# Autodesk Inventor assembly: LED Assembly
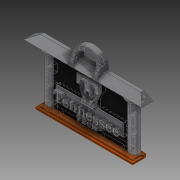
[picture p0: Inventor's stored thumbnail of the model, 180x180]
Saved by Autodesk Inventor 2018 (Build 220112000, 112)
## iProperties
Created: 2017-12-07
Part Number: LED Assembly
Document SubType Name: Assembly
Designer: Rus
Author: Rus
## Documents named in this file (10)
- E:\Libraries\Documents\3D Models\2017 TN Tech Ornament\Split\LED Assembly SPLIT.iam
- E:\Libraries\Documents\3D Models\2017 TN Tech Ornament\LED.ipt
- E:\Libraries\Documents\3D Models\2017 TN Tech Ornament\Split\3D Printed2 LED parent.ipt
- E:\Libraries\Documents\3D Models\2017 TN Tech Ornament\Split\3D Printed2 LED Pillar R white.ipt
- E:\Libraries\Documents\3D Models\2017 TN Tech Ornament\Split\3D Printed2 LED Top Grey.ipt
- E:\Libraries\Documents\3D Models\2017 TN Tech Ornament\Split\3D Printed2 LED Pillar L white 2.ipt
- E:\Libraries\Documents\3D Models\2017 TN Tech Ornament\Split\3D Printed2 LED Steps Brown.ipt
- E:\Libraries\Documents\3D Models\2017 TN Tech Ornament\Split\3D Printed2 LED Mid Black.ipt
- E:\Libraries\Documents\3D Models\2017 TN Tech Ornament\Split\3D Printed2 LED Text Bird.ipt
- E:\Libraries\Documents\3D Models\2017 TN Tech Ornament\Split\3D Printed2 LED Text text.ipt
## Components (18 placed, 9 different names)
1. LED:1 — Angle:2, Angle:18, Insert:1
2. 3D Printed2 LED parent:1 — Angle:2, Angle:3, Angle:4, Angle:5, Angle:6, Angle:7, Angle:8, Angle:9, Angle:10, Angle:11, Angle:12, Angle:13, Angle:14, Angle:15, Angle:16, Angle:17, Angle:18, Insert:1, Insert:2, Insert:3, Insert:4, Insert:5, Insert:6, Insert:7, Insert:8, Insert:9, Insert:10
3. LED:2 — Angle:4, Angle:16, Insert:4
4. LED:3 — Angle:5, Angle:15, Insert:2
5. LED:4 — Angle:3, Angle:17, Insert:6
6. LED:5 — Angle:9, Insert:9
7. LED:6 — Angle:7, Angle:13, Insert:3
8. LED:7 — Angle:8, Angle:11, Insert:7
9. LED:8 — Angle:6, Angle:14, Insert:8
10. LED:9 — Angle:10, Insert:5
11. LED:10 — Angle:12, Insert:10
12. 3D Printed2 LED Pillar R white:1 — Flush:2, Mate:1, Mate:3, Flush:3, Flush:4, Flush:6, Mate:8
13. 3D Printed2 LED Top Grey:1 — Flush:2, Mate:1, Mate:2, Angle:19, Mate:4, Mate:6, Angle:21, Mate:11, Angle:22, Mate:14
14. 3D Printed2 LED Pillar L white 2:1 — Flush:3, Flush:4, Mate:4, Flush:7, Flush:9
15. 3D Printed2 LED Steps Brown:1 — Flush:6, Mate:8, Flush:7
16. 3D Printed2 LED Mid Black:1 — Flush:8, Mate:9, Mate:10, Flush:9, Mate:12, Angle:23, Mate:14
17. 3D Printed2 LED Text Bird:1 — Flush:8, Mate:9, Mate:10
18. 3D Printed2 LED Text text:1
## Relationships (51: Angle 21, Mate 13, Insert 10, Flush 7)
- Angle:2 (0 deg): LED:1 ↔ 3D Printed2 LED parent:1
- Angle:3 (0 deg): 3D Printed2 LED parent:1 ↔ LED:4
- Angle:4 (0 deg): 3D Printed2 LED parent:1 ↔ LED:2
- Angle:5 (0 deg): 3D Printed2 LED parent:1 ↔ LED:3
- Angle:6 (0 deg): 3D Printed2 LED parent:1 ↔ LED:8
- Angle:7 (0 deg): 3D Printed2 LED parent:1 ↔ LED:6
- Angle:8 (0 deg): 3D Printed2 LED parent:1 ↔ LED:7
- Angle:9 (0 deg): 3D Printed2 LED parent:1 ↔ LED:5
- Angle:10 (0 deg): 3D Printed2 LED parent:1 ↔ LED:9
- Angle:11 (0 deg): 3D Printed2 LED parent:1 ↔ LED:7
- Angle:12 (0 deg): 3D Printed2 LED parent:1 ↔ LED:10
- Angle:13 (0 deg): 3D Printed2 LED parent:1 ↔ LED:6
- Angle:14 (0 deg): 3D Printed2 LED parent:1 ↔ LED:8
- Angle:15 (0 deg): 3D Printed2 LED parent:1 ↔ LED:3
- Angle:16 (0 deg): 3D Printed2 LED parent:1 ↔ LED:2
- Angle:17 (0 deg): 3D Printed2 LED parent:1 ↔ LED:4
- Angle:18 (0 deg): LED:1 ↔ 3D Printed2 LED parent:1
- Insert:1: LED:1 ↔ 3D Printed2 LED parent:1
- Insert:2: 3D Printed2 LED parent:1 ↔ LED:3
- Insert:3: 3D Printed2 LED parent:1 ↔ LED:6
- Insert:4: 3D Printed2 LED parent:1 ↔ LED:2
- Insert:5: 3D Printed2 LED parent:1 ↔ LED:9
- Insert:6: 3D Printed2 LED parent:1 ↔ LED:4
- Insert:7: 3D Printed2 LED parent:1 ↔ LED:7
- Insert:8: 3D Printed2 LED parent:1 ↔ LED:8
- Insert:9: 3D Printed2 LED parent:1 ↔ LED:5
- Insert:10: 3D Printed2 LED parent:1 ↔ LED:10
- Flush:2: 3D Printed2 LED Pillar R white:1 ↔ 3D Printed2 LED Top Grey:1
- Mate:1: 3D Printed2 LED Pillar R white:1 ↔ 3D Printed2 LED Top Grey:1
- Mate:2: 3D Printed2 LED Top Grey:1
- Angle:19 (0 deg): 3D Printed2 LED Top Grey:1
- Mate:3 (33.8667 mm): 3D Printed2 LED Pillar R white:1
- Flush:3: 3D Printed2 LED Pillar R white:1 ↔ 3D Printed2 LED Pillar L white 2:1
- Flush:4: 3D Printed2 LED Pillar R white:1 ↔ 3D Printed2 LED Pillar L white 2:1
- Mate:4: 3D Printed2 LED Top Grey:1 ↔ 3D Printed2 LED Pillar L white 2:1
- Flush:6: 3D Printed2 LED Pillar R white:1 ↔ 3D Printed2 LED Steps Brown:1
- Mate:6: 3D Printed2 LED Top Grey:1
- Angle:21 (0 deg): 3D Printed2 LED Top Grey:1
- Mate:7
- Mate:8: 3D Printed2 LED Pillar R white:1 ↔ 3D Printed2 LED Steps Brown:1
- Flush:7: 3D Printed2 LED Pillar L white 2:1 ↔ 3D Printed2 LED Steps Brown:1
- Flush:8: 3D Printed2 LED Mid Black:1 ↔ 3D Printed2 LED Text Bird:1
- Mate:9: 3D Printed2 LED Mid Black:1 ↔ 3D Printed2 LED Text Bird:1
- Mate:10: 3D Printed2 LED Mid Black:1 ↔ 3D Printed2 LED Text Bird:1
- Flush:9: 3D Printed2 LED Pillar L white 2:1 ↔ 3D Printed2 LED Mid Black:1
- Mate:11: 3D Printed2 LED Top Grey:1
- Angle:22 (0 deg): 3D Printed2 LED Top Grey:1
- Mate:12: 3D Printed2 LED Mid Black:1
- Angle:23 (0 deg): 3D Printed2 LED Mid Black:1
- Mate:13
- Mate:14: 3D Printed2 LED Top Grey:1 ↔ 3D Printed2 LED Mid Black:1
